# Autodesk Inventor assembly: FeederV2
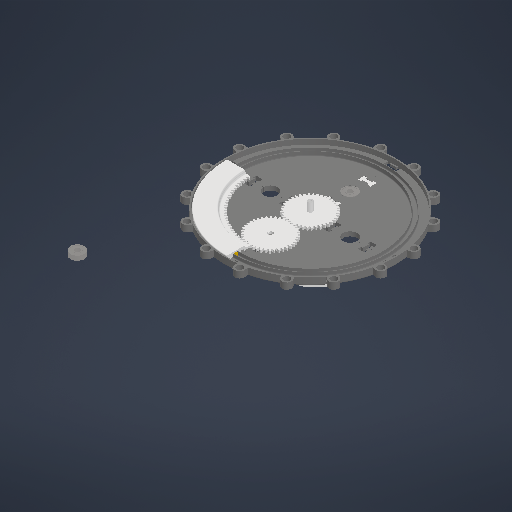
[picture p0: Inventor's stored thumbnail of the model, 512x512]
Saved by Autodesk Inventor 2026 (Build 300175050, 175E)
## iProperties
Created: 2026-03-26
Part Number: FeederV2
Document SubType Name: Assembly
Designer: sniel
Author: sniel
## Documents named in this file (27)
- C:\Users\sniel\OneDrive\SDU\4_Semester\Applied automation\AppliedAutomationProject\feeder\FeederV2.iam
- C:\Users\sniel\OneDrive\SDU\4_Semester\Applied automation\AppliedAutomationProject\feeder\base plate.ipt
- C:\Users\sniel\OneDrive\SDU\4_Semester\Applied automation\AppliedAutomationProject\feeder\outerspinnerV3.ipt
- C:\Users\sniel\OneDrive\SDU\4_Semester\Applied automation\AppliedAutomationProject\feeder\gears1.ipt
- C:\Users\sniel\OneDrive\SDU\4_Semester\Applied automation\AppliedAutomationProject\feeder\FeederV2\Design Accelerator\Spur Gears5.iam
- C:\Users\sniel\OneDrive\SDU\4_Semester\Applied automation\AppliedAutomationProject\feeder\centrer centrifugal spinner.ipt
- C:\Users\sniel\OneDrive\SDU\4_Semester\Applied automation\AppliedAutomationProject\feeder\central axel.ipt
- C:\Users\sniel\OneDrive\SDU\4_Semester\Applied automation\AppliedAutomationProject\feeder\base frame.ipt
- C:\Users\sniel\OneDrive\SDU\4_Semester\Applied automation\AppliedAutomationProject\feeder\moon_gear_V1.ipt
- C:\Users\sniel\OneDrive\SDU\4_Semester\Applied automation\AppliedAutomationProject\feeder\primlock.ipt
- C:\Users\sniel\OneDrive\SDU\4_Semester\Applied automation\AppliedAutomationProject\feeder\outerdisk_pin.ipt
- C:\Users\sniel\OneDrive\SDU\4_Semester\Applied automation\AppliedAutomationProject\feeder\roll_ball_1.ipt
- C:\Users\sniel\OneDrive\SDU\4_Semester\Applied automation\AppliedAutomationProject\feeder\Leg_v1.ipt
- C:\Users\sniel\OneDrive\SDU\4_Semester\Applied automation\AppliedAutomationProject\feeder\main axel.ipt
- C:\Users\sniel\OneDrive\fritid\3D print\s-Toy\Plug\STL\ServoMotor.ipt
- C:\Users\sniel\OneDrive\SDU\4_Semester\Applied automation\AppliedAutomationProject\feeder\Base_frame_v2.ipt
- C:\Users\sniel\OneDrive\SDU\4_Semester\Applied automation\AppliedAutomationProject\feeder\Metal bearing.ipt
- C:\Users\sniel\OneDrive\SDU\4_Semester\Applied automation\AppliedAutomationProject\feeder\outerspinner_v3.ipt
- C:\Users\sniel\OneDrive\SDU\4_Semester\Applied automation\AppliedAutomationProject\feeder\FeederV2\Design Accelerator\Spur Gears11.iam
- C:\Users\sniel\OneDrive\SDU\4_Semester\Applied automation\AppliedAutomationProject\feeder\Central_axel_Gear.ipt
- C:\Users\sniel\OneDrive\SDU\4_Semester\Applied automation\AppliedAutomationProject\feeder\moon_gear_v2.ipt
- C:\Users\sniel\OneDrive\SDU\4_Semester\Applied automation\AppliedAutomationProject\feeder\halfAxel.ipt
- C:\Users\sniel\OneDrive\SDU\4_Semester\Applied automation\AppliedAutomationProject\feeder\TopSpinner_steep_angle_V2.ipt
- C:\Users\sniel\OneDrive\SDU\4_Semester\Applied automation\AppliedAutomationProject\feeder\STEP\45angleBase.ipt
- C:\Users\sniel\OneDrive\SDU\4_Semester\Applied automation\AppliedAutomationProject\feeder\FeederV2\Design Accelerator\Bevel Gears1.iam
- C:\Users\sniel\OneDrive\SDU\4_Semester\Applied automation\AppliedAutomationProject\feeder\FeederV2\Design Accelerator\Bevel Gears2.iam
- C:\Users\sniel\OneDrive\SDU\4_Semester\Applied automation\AppliedAutomationProject\feeder\FeederV2\Design Accelerator\Bevel Gears3.iam
## Components (32 placed, 23 different names)
1. base plate:1
2. outerspinnerV3:1 — Mate:1, Mate:2, Mate:3, Mate:4, Flush:2, Mate:6
3. gears1:1 — Mate:3
4. Spur Gears:4 [sub-assembly] — Mate:1, Mate:2
5. centrer centrifugal spinner:1 — Mate:4, Flush:1
6. central axel:1 — Flush:1, Mate:5, Flush:4
7. base frame:1 — Mate:5, Flush:2, Mate:6, Mate:7, Mate:8, Mate:9, Mate:11, Mate:12, Mate:13, Mate:14
8. moon_gear_V1:1 — Mate:7, Mate:8, Mate:10, Flush:3
9. moon_gear_V1:2 — Mate:9, Mate:11
10. primlock:1 — Mate:10, Flush:3
11. outerdisk_pin:1 — Mate:12
12. roll_ball_1:1
13. Leg_v1:1 — Mate:13, Mate:14
14. main axel:1 — Flush:4
15. ServoMotor:1 — Mate:15, Mate:16, Mate:17
16. Base_frame_v2:1 — Mate:15, Mate:16, Mate:17, Mate:18, Mate:19, Flush:7, Mate:20, Mate:22, Mate:23, Mate:24, Flush:8, Mate:26, Flush:9, Flush:10, Mate:28, Flush:13, Mate:29
17. Metal bearing:1
18. outerspinner_v3:1 — Mate:18, Mate:23, Flush:8
19. Spur Gears:5 [sub-assembly]
20. Central_axel_Gear:1 — Mate:19, Mate:20
21. moon_gear_v2:1 — Flush:7, Mate:22
22. Metal bearing:2 — Mate:24, Mate:25
23. halfAxel:1 — Mate:25
24. TopSpinner_steep_angle_V2:1
25. Base_frame_v2:2 — Mate:26, Flush:9, Flush:10, Mate:30, Mate:31, Flush:14, Mate:32, Flush:15
26. Base_frame_v2:3
27. Base_frame_v2:4 — Mate:28, Flush:13, Mate:29
28. 45angleBase:1 — Mate:30, Mate:31, Flush:14
29. Metal bearing:3 — Mate:32, Flush:15
30. Bevel Gears:1 [sub-assembly]
31. Bevel Gears:2 [sub-assembly]
32. Bevel Gears:3 [sub-assembly]
## Relationships (44: Mate 31, Flush 13)
- Mate:1: outerspinnerV3:1 ↔ Spur Gears:4
- Mate:2: outerspinnerV3:1 ↔ Spur Gears:4
- Mate:3: outerspinnerV3:1 ↔ gears1:1
- Mate:4: outerspinnerV3:1 ↔ centrer centrifugal spinner:1
- Flush:1: centrer centrifugal spinner:1 ↔ central axel:1
- Mate:5: central axel:1 ↔ base frame:1
- Flush:2: outerspinnerV3:1 ↔ base frame:1
- Mate:6: outerspinnerV3:1 ↔ base frame:1
- Mate:7: base frame:1 ↔ moon_gear_V1:1
- Mate:8: base frame:1 ↔ moon_gear_V1:1
- Mate:9: base frame:1 ↔ moon_gear_V1:2
- Mate:10: moon_gear_V1:1 ↔ primlock:1
- Flush:3: moon_gear_V1:1 ↔ primlock:1
- Mate:11: base frame:1 ↔ moon_gear_V1:2
- Mate:12: base frame:1 ↔ outerdisk_pin:1
- Mate:13: base frame:1 ↔ Leg_v1:1
- Mate:14: base frame:1 ↔ Leg_v1:1
- Flush:4: central axel:1 ↔ main axel:1
- Mate:15: ServoMotor:1 ↔ Base_frame_v2:1
- Mate:16: ServoMotor:1 ↔ Base_frame_v2:1
- Mate:17: ServoMotor:1 ↔ Base_frame_v2:1
- Mate:18: Base_frame_v2:1 ↔ outerspinner_v3:1
- Mate:19: Base_frame_v2:1 ↔ Central_axel_Gear:1
- Flush:7 (1 mm): Base_frame_v2:1 ↔ moon_gear_v2:1
- Mate:20 (1 mm): Base_frame_v2:1 ↔ Central_axel_Gear:1
- Mate:22: Base_frame_v2:1 ↔ moon_gear_v2:1
- Mate:23 (1 mm): Base_frame_v2:1 ↔ outerspinner_v3:1
- Mate:24: Base_frame_v2:1 ↔ Metal bearing:2
- Mate:25: Metal bearing:2 ↔ halfAxel:1
- Flush:8: Base_frame_v2:1 ↔ outerspinner_v3:1
- Mate:26: Base_frame_v2:1 ↔ Base_frame_v2:2
- Flush:9: Base_frame_v2:1 ↔ Base_frame_v2:2
- Flush:10: Base_frame_v2:1 ↔ Base_frame_v2:2
- [Mate]: Base_frame_v2:3 ↔ Base_frame_v2:4
- [Flush]: Base_frame_v2:3 ↔ Base_frame_v2:4
- [Flush]: Base_frame_v2:3 ↔ Base_frame_v2:4
- Mate:28: Base_frame_v2:1 ↔ Base_frame_v2:4
- Flush:13: Base_frame_v2:1 ↔ Base_frame_v2:4
- Mate:29: Base_frame_v2:1 ↔ Base_frame_v2:4
- Mate:30 (0.15 mm): Base_frame_v2:2 ↔ 45angleBase:1
- Mate:31 (0.15 mm): Base_frame_v2:2 ↔ 45angleBase:1
- Flush:14: Base_frame_v2:2 ↔ 45angleBase:1
- Mate:32: Base_frame_v2:2 ↔ Metal bearing:3
- Flush:15: Base_frame_v2:2 ↔ Metal bearing:3
## Named parameters: d53_d52 = 0 mm, d54_d50 = 0 mm, d55_d51 = 0 mm
